# Autodesk Inventor assembly: X Axis
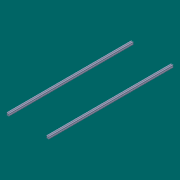
[picture p0: Inventor's stored thumbnail of the model, 180x180]
Saved by Autodesk Inventor 2016 (Build 200138000, 138)
## iProperties
Created: 2015-06-02
Part Number: X Axis
Document SubType Name: Assembly
Designer: Sawaiz Syed
Author: Sawaiz Syed
## Documents named in this file (2)
- C:\Users\Sawaiz\Documents\data\projects\cncBlackBox\xAxis\xAxis.iam
- C:\Users\Sawaiz\Documents\data\projects\cncBlackBox\xAxis\xAxisVslot.ipt
## Components (2 placed, 1 different names)
1. xAxisVslot:1 — Flush:3, Flush:4, Flush:7
2. xAxisVslot:2 — Flush:3, Flush:4, Flush:7
## Relationships (5: Flush 5)
- [Flush]: xAxisVslot:1 ↔ xAxisVslot:2
- [Flush]: xAxisVslot:1 ↔ xAxisVslot:2
- Flush:3: xAxisVslot:1 ↔ xAxisVslot:2
- Flush:4: xAxisVslot:1 ↔ xAxisVslot:2
- Flush:7 (-320 mm): xAxisVslot:1 ↔ xAxisVslot:2
